# Autodesk Inventor assembly: horn_v0.1
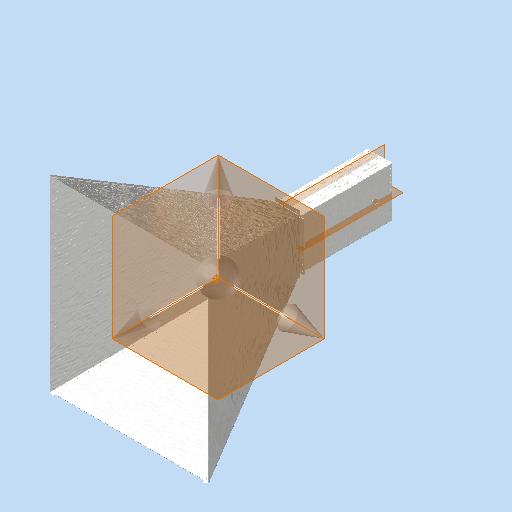
[picture p0: Inventor's stored thumbnail of the model, 512x512]
Saved by Autodesk Inventor 2026.2 (Build 302298000, 298)
## iProperties
Created: 2026-02-28
Part Number: horn_v0.1
Document SubType Name: Assembly
Designer: alpgo
Mass: 3918.18 g
Surface Area: 19620.5 cm^2
Volume: 1462.01 cm^3
Density: 2.68 g/cm^3
Author: alpgo
## Documents named in this file (5)
- C:\Users\alpgo\OneDrive\Documents\Inventor\horn type shii\horn goats\horn_v0.1.iam
- C:\Users\alpgo\OneDrive\Documents\Inventor\horn type shii\horn goats\hplane_v0.3.ipt
- C:\Users\alpgo\OneDrive\Documents\Inventor\horn type shii\horn goats\eplane_v0.3.ipt
- C:\Users\alpgo\OneDrive\Documents\Inventor\horn type shii\horn goats\wave_0.1.ipt
- C:\Users\alpgo\OneDrive\Documents\Inventor\horn type shii\horn goats\backshort_0.1.ipt
## Components (6 placed, 4 different names)
1. hplane_v0.3:1 — Mate:1, Mate:2, Mate:3, Mate:4, Mate:5, Mate:6, Mate:7, Mate:8
2. eplane_v0.3:1 — Mate:1, Mate:2, Mate:3
3. eplane_v0.3:2 — Mate:6, Mate:7, Mate:8, Mate:9, Mate:10, Mate:11, Mate:12, Mate:13, Mate:14
4. hplane_v0.3:2 — Mate:9, Mate:10, Mate:11
5. wave_0.1:1 — Mate:12, Mate:13, Mate:14, Mate:15, Mate:16, Mate:17
6. backshort_0.1:1 — Mate:15, Mate:16, Mate:17
## Relationships (17: Mate 17)
- Mate:1: hplane_v0.3:1 ↔ eplane_v0.3:1
- Mate:2: hplane_v0.3:1 ↔ eplane_v0.3:1
- Mate:3: hplane_v0.3:1 ↔ eplane_v0.3:1
- Mate:4: hplane_v0.3:1
- Mate:5: hplane_v0.3:1
- Mate:6: hplane_v0.3:1 ↔ eplane_v0.3:2
- Mate:7: hplane_v0.3:1 ↔ eplane_v0.3:2
- Mate:8: hplane_v0.3:1 ↔ eplane_v0.3:2
- Mate:9: eplane_v0.3:2 ↔ hplane_v0.3:2
- Mate:10: eplane_v0.3:2 ↔ hplane_v0.3:2
- Mate:11: eplane_v0.3:2 ↔ hplane_v0.3:2
- Mate:12: eplane_v0.3:2 ↔ wave_0.1:1
- Mate:13: eplane_v0.3:2 ↔ wave_0.1:1
- Mate:14: eplane_v0.3:2 ↔ wave_0.1:1
- Mate:15: wave_0.1:1 ↔ backshort_0.1:1
- Mate:16: wave_0.1:1 ↔ backshort_0.1:1
- Mate:17: wave_0.1:1 ↔ backshort_0.1:1
